# Autodesk Inventor assembly: Assembly1
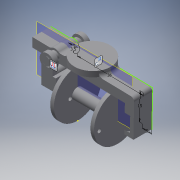
[picture p0: Inventor's stored thumbnail of the model, 180x180]
Saved by Autodesk Inventor 2019 (Build 230136000, 136)
## iProperties
Created: 2019-01-13
Part Number: Assembly1
Document SubType Name: Assembly
Designer: Kepler
Author: Kepler
## Documents named in this file (5)
- C:\Users\Kepler\Documents\Inventor\Organ Valves\Assembly1.iam
- C:\Users\Kepler\Documents\Inventor\Organ Valves\SpoolNoCenterHole1.ipt
- C:\Users\Kepler\Documents\Inventor\Organ Valves\Rocker1.ipt
- C:\Users\Kepler\Documents\Inventor\Organ Valves\HingeBase1.ipt
- C:\Users\Kepler\Documents\Inventor\Organ Valves\Axle 1.ipt
## Components (4 placed, 4 different names)
1. SpoolNoCenterHole1:1 — Mate:2, Mate:3
2. Rocker1:1 — Mate:1, Angle:1, Insert:1
3. HingeBase1:1 — Mate:2, Insert:2, Mate:3
4. Axle 1:1 — Insert:1, Insert:2
## Relationships (6: Mate 3, Insert 2, Angle 1)
- Mate:1: Rocker1:1
- Angle:1 (0 deg): Rocker1:1
- Insert:1 (-15 mm): Rocker1:1 ↔ Axle 1:1
- Mate:2: SpoolNoCenterHole1:1 ↔ HingeBase1:1
- Insert:2 (-20 mm): HingeBase1:1 ↔ Axle 1:1
- Mate:3: SpoolNoCenterHole1:1 ↔ HingeBase1:1
